# Autodesk Inventor assembly: robot
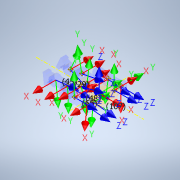
[picture p0: Inventor's stored thumbnail of the model, 180x180]
Saved by Autodesk Inventor 2020.2 (Build 242310000, 310)
## iProperties
Created: 2021-01-29
Part Number: robot
Document SubType Name: Assembly
Designer: DELL
Author: DELL
## Documents named in this file (9)
- D:\repo\FlexipodFast\robot\v11\mesh\robot.iam
- D:\repo\FlexipodFast\robot\v11\mesh\hip.ipt
- D:\repo\FlexipodFast\robot\v11\mesh\thigh.ipt
- D:\repo\FlexipodFast\robot\v11\mesh\shank_back.ipt
- D:\repo\FlexipodFast\robot\v11\mesh\shank_front.ipt
- D:\repo\FlexipodFast\robot\v11\mesh\body.ipt
- D:\repo\FlexipodFast\robot\v11\mesh\shank_back_mirror.ipt
- D:\repo\FlexipodFast\robot\v11\mesh\hip_back.ipt
- D:\repo\FlexipodFast\robot\v11\mesh\knee.ipt
## Components (13 placed, 8 different names)
1. hip:1 — Rotational:1, Angle:34, Rotational:11
2. hip:2 — Rotational:2, Rotational:9, Angle:33
3. thigh:1 — Rotational:9, Rotational:15
4. thigh:2 — Rotational:10, Rotational:11
5. shank_back:3 — Angle:37, Rotational:23
6. shank_front:1 — Rotational:10
7. shank_front:2 — Rotational:15
8. body:1 — Flush:47, Flush:48, Flush:49, Rotational:1, Rotational:2, Angle:33, Angle:34, Angle:37, Rotational:19, Rotational:24
9. shank_back_mirror:1 — Rotational:21
10. hip_back:1 — Rotational:22, Rotational:24
11. hip_back:2 — Rotational:19, Rotational:20
12. knee:1 — Rotational:20, Rotational:21
13. knee:4 — Rotational:22, Rotational:23
## Relationships (18: RevoluteJoint 12, Flush 3, Angle 3)
- Flush:47: body:1
- Flush:48: body:1
- Flush:49: body:1
- Rotational:1 [RevoluteJoint]: hip:1 ↔ body:1
- Rotational:2 [RevoluteJoint]: hip:2 ↔ body:1
- Rotational:9 [RevoluteJoint]: hip:2 ↔ thigh:1
- Angle:33 (0 deg): hip:2 ↔ body:1
- Angle:34 (180 deg): hip:1 ↔ body:1
- Rotational:10 [RevoluteJoint]: thigh:2 ↔ shank_front:1
- Rotational:11 [RevoluteJoint]: hip:1 ↔ thigh:2
- Rotational:15 [RevoluteJoint]: thigh:1 ↔ shank_front:2
- Angle:37 (0 deg): shank_back:3 ↔ body:1
- Rotational:19 [RevoluteJoint]: body:1 ↔ hip_back:2
- Rotational:20 [RevoluteJoint]: hip_back:2 ↔ knee:1
- Rotational:21 [RevoluteJoint]: shank_back_mirror:1 ↔ knee:1
- Rotational:22 [RevoluteJoint]: hip_back:1 ↔ knee:4
- Rotational:23 [RevoluteJoint]: shank_back:3 ↔ knee:4
- Rotational:24 [RevoluteJoint]: body:1 ↔ hip_back:1
